# Autodesk Inventor assembly: Grid_Of_Piers
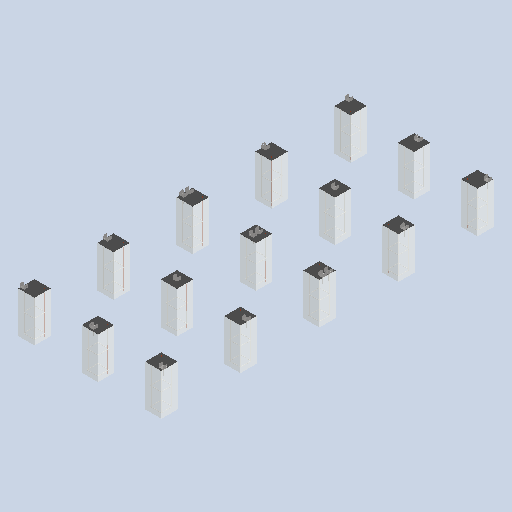
[picture p0: Inventor's stored thumbnail of the model, 512x512]
Saved by Autodesk Inventor 2025.1 (Build 291241020, 241B)
## iProperties
Created: 2024-08-07
Part Number: Grid_Of_Piers
Document SubType Name: Assembly
Designer: Tom
Author: Tom
## Documents named in this file (4)
- C:\Users\Tom\Documents\Inventor\Mobility\Additional_Building\Grid_Of_Piers.iam
- C:\Users\Tom\Documents\Inventor\Mobility\Additional_Building\Pier.iam
- C:\Users\Tom\Documents\Inventor\Mobility\Additional_Building\Saddle_Bracket.ipt
- C:\Users\Tom\Documents\Inventor\Mobility\Additional_Building\Ground_Rod.ipt
## Components (48 placed, 3 different names)
1. Saddle_Bracket:1 — Mate:1, Flush:1, Flush:2
2. Saddle_Bracket:2 — Mate:2, Flush:3, Mate:10
3. Saddle_Bracket:3 — Mate:3, Flush:5, Mate:11
4. Saddle_Bracket:4 — Mate:4, Flush:7, Mate:12
5. Saddle_Bracket:5 — Mate:5, Mate:6, Mate:7
6. Saddle_Bracket:6 — Mate:8, Mate:9, Mate:13
7. Saddle_Bracket:7 — Mate:14, Flush:8, Flush:9
8. Saddle_Bracket:8 — Mate:15, Flush:10, Mate:16
9. Saddle_Bracket:9 — Flush:11, Mate:17, Flush:12
10. Saddle_Bracket:10 — Mate:18, Mate:19, Flush:13
11. Saddle_Bracket:11 — Mate:20, Mate:21, Mate:22
12. Saddle_Bracket:12 — Mate:23, Flush:14, Mate:24
13. Saddle_Bracket:13 — Mate:25, Flush:15, Flush:18
14. Saddle_Bracket:14 — Mate:27, Mate:28, Flush:17
15. Saddle_Bracket:15 — Mate:30, Mate:31, Flush:16
16. Saddle_Bracket:16 — Mate:32, Mate:33, Flush:21
17. Saddle_Bracket:17 — Mate:35, Flush:19, Flush:20
18. Saddle_Bracket:18 — Mate:36, Flush:22, Flush:23
19. Ground_Rod:1 — Flush:24, Tangent:1, Tangent:2
20. Ground_Rod:2 — Flush:25, Tangent:3, Tangent:4
21. Ground_Rod:3 — Flush:26, Tangent:5, Tangent:6
22. Ground_Rod:4 — Flush:27, Mate:40, Mate:41
23. Ground_Rod:5 — Flush:28, Mate:45, Mate:46
24. Ground_Rod:6 — Flush:29, Mate:47, Mate:48
25. Ground_Rod:7 — Flush:30, Mate:53, Mate:54
26. Ground_Rod:8 — Flush:31, Mate:44, Flush:41
27. Ground_Rod:9 — Flush:32, Mate:43, Flush:40
28. Ground_Rod:10 — Flush:33, Tangent:7, Tangent:9, Tangent:10
29. Ground_Rod:11 — Flush:34, Mate:42, Flush:39
30. Ground_Rod:12 — Flush:35, Mate:49, Mate:50
31. Ground_Rod:13 — Flush:36, Mate:51, Mate:52
32. Ground_Rod:14 — Flush:37, Mate:55, Flush:42
33. Ground_Rod:15 — Flush:38, Mate:56, Flush:43
34. Pier:1 [sub-assembly] — Mate:1, Flush:1, Flush:2, Mate:37, Mate:38, Mate:39, Flush:28, Mate:40, Mate:41
35. Pier:2 [sub-assembly] — Mate:2, Flush:3, Mate:10, Flush:27, Tangent:7, Tangent:9, Tangent:10
36. Pier:3 [sub-assembly] — Mate:3, Flush:5, Mate:11, Mate:14, Flush:8, Flush:9, Flush:26, Tangent:5, Tangent:6
37. Pier:4 [sub-assembly] — Mate:15, Flush:10, Mate:16, Flush:25, Tangent:3, Tangent:4
38. Pier:5 [sub-assembly] — Flush:11, Mate:17, Flush:12, Flush:24, Tangent:1, Tangent:2
39. Pier:6 [sub-assembly] — Mate:4, Flush:7, Mate:12, Flush:29, Mate:47, Mate:48
40. Pier:7 [sub-assembly] — Mate:5, Mate:6, Mate:7, Flush:30, Mate:45, Mate:46
41. Pier:8 [sub-assembly] — Mate:8, Mate:9, Mate:13, Mate:18, Mate:19, Flush:13, Flush:31, Mate:44, Flush:41
42. Pier:9 [sub-assembly] — Mate:20, Mate:21, Mate:22, Flush:32, Mate:43, Flush:40
43. Pier:10 [sub-assembly] — Mate:23, Flush:14, Mate:24, Flush:33, Mate:42, Flush:39
44. Pier:11 [sub-assembly] — Mate:25, Flush:15, Flush:18, Flush:38, Mate:56, Flush:43
45. Pier:12 [sub-assembly] — Mate:27, Mate:28, Flush:17, Flush:37, Mate:55, Flush:42
46. Pier:13 [sub-assembly] — Mate:30, Mate:31, Flush:16, Mate:36, Flush:22, Flush:23, Flush:36, Mate:53, Mate:54
47. Pier:14 [sub-assembly] — Mate:32, Mate:33, Flush:21, Flush:35, Mate:51, Mate:52
48. Pier:15 [sub-assembly] — Mate:35, Flush:19, Flush:20, Flush:34, Mate:49, Mate:50
## Component patterns: (15 elements, first: Pier:1)
## Relationships (103: Mate 53, Flush 41, Tangent 9)
- Mate:1: Saddle_Bracket:1 ↔ Pier:1
- Flush:1 (-3.175 mm): Saddle_Bracket:1 ↔ Pier:1
- Flush:2 (38.1 mm): Saddle_Bracket:1 ↔ Pier:1
- Mate:2: Saddle_Bracket:2 ↔ Pier:2
- Flush:3 (-3.175 mm): Saddle_Bracket:2 ↔ Pier:2
- Mate:3: Saddle_Bracket:3 ↔ Pier:3
- Flush:5 (-3.175 mm): Saddle_Bracket:3 ↔ Pier:3
- Mate:4: Saddle_Bracket:4 ↔ Pier:6
- Flush:7 (38.1 mm): Saddle_Bracket:4 ↔ Pier:6
- Mate:5: Saddle_Bracket:5 ↔ Pier:7
- Mate:6: Saddle_Bracket:5 ↔ Pier:7
- Mate:7: Saddle_Bracket:5 ↔ Pier:7
- Mate:8: Saddle_Bracket:6 ↔ Pier:8
- Mate:9: Saddle_Bracket:6 ↔ Pier:8
- Mate:10: Saddle_Bracket:2 ↔ Pier:2
- Mate:11 (19.05 mm): Saddle_Bracket:3 ↔ Pier:3
- Mate:12: Saddle_Bracket:4 ↔ Pier:6
- Mate:13 (19.05 mm): Saddle_Bracket:6 ↔ Pier:8
- Mate:14: Saddle_Bracket:7 ↔ Pier:3
- Flush:8 (-3.175 mm): Saddle_Bracket:7 ↔ Pier:3
- Flush:9 (19.05 mm): Saddle_Bracket:7 ↔ Pier:3
- Mate:15: Saddle_Bracket:8 ↔ Pier:4
- Flush:10 (-3.175 mm): Saddle_Bracket:8 ↔ Pier:4
- Mate:16: Saddle_Bracket:8 ↔ Pier:4
- Flush:11 (38.1 mm): Saddle_Bracket:9 ↔ Pier:5
- Mate:17: Saddle_Bracket:9 ↔ Pier:5
- Flush:12 (-3.175 mm): Saddle_Bracket:9 ↔ Pier:5
- Mate:18: Saddle_Bracket:10 ↔ Pier:8
- Mate:19: Saddle_Bracket:10 ↔ Pier:8
- Flush:13 (19.05 mm): Saddle_Bracket:10 ↔ Pier:8
- Mate:20: Saddle_Bracket:11 ↔ Pier:9
- Mate:21: Saddle_Bracket:11 ↔ Pier:9
- Mate:22: Saddle_Bracket:11 ↔ Pier:9
- Mate:23: Saddle_Bracket:12 ↔ Pier:10
- Flush:14 (38.1 mm): Saddle_Bracket:12 ↔ Pier:10
- Mate:24: Saddle_Bracket:12 ↔ Pier:10
- Mate:25: Saddle_Bracket:13 ↔ Pier:11
- Flush:15 (38.1 mm): Saddle_Bracket:13 ↔ Pier:11
- Mate:27: Saddle_Bracket:14 ↔ Pier:12
- Mate:28: Saddle_Bracket:14 ↔ Pier:12
- Mate:30: Saddle_Bracket:15 ↔ Pier:13
- Mate:31 (19.05 mm): Saddle_Bracket:15 ↔ Pier:13
- Flush:16 (-3.175 mm): Saddle_Bracket:15 ↔ Pier:13
- Flush:17 (-3.175 mm): Saddle_Bracket:14 ↔ Pier:12
- Flush:18 (-3.175 mm): Saddle_Bracket:13 ↔ Pier:11
- Mate:32: Saddle_Bracket:16 ↔ Pier:14
- Mate:33: Saddle_Bracket:16 ↔ Pier:14
- Mate:35: Saddle_Bracket:17 ↔ Pier:15
- Flush:19 (-3.175 mm): Saddle_Bracket:17 ↔ Pier:15
- Flush:20 (38.1 mm): Saddle_Bracket:17 ↔ Pier:15
- Flush:21 (-3.175 mm): Saddle_Bracket:16 ↔ Pier:14
- Mate:36: Saddle_Bracket:18 ↔ Pier:13
- Flush:22 (-3.175 mm): Saddle_Bracket:18 ↔ Pier:13
- Flush:23 (19.05 mm): Saddle_Bracket:18 ↔ Pier:13
- Mate:37: Pier:1
- Mate:38: Pier:1
- Mate:39: Pier:1
- Flush:24 (-12.7 mm): Ground_Rod:1 ↔ Pier:5
- Flush:25 (-12.7 mm): Ground_Rod:2 ↔ Pier:4
- Flush:26 (-12.7 mm): Ground_Rod:3 ↔ Pier:3
- Flush:27 (-12.7 mm): Ground_Rod:4 ↔ Pier:2
- Flush:28 (-12.7 mm): Ground_Rod:5 ↔ Pier:1
- Flush:29 (-12.7 mm): Ground_Rod:6 ↔ Pier:6
- Flush:30 (-12.7 mm): Ground_Rod:7 ↔ Pier:7
- Flush:31 (-12.7 mm): Ground_Rod:8 ↔ Pier:8
- Flush:32 (-12.7 mm): Ground_Rod:9 ↔ Pier:9
- Flush:33 (-12.7 mm): Ground_Rod:10 ↔ Pier:10
- Flush:34 (-12.7 mm): Ground_Rod:11 ↔ Pier:15
- Flush:35 (-12.7 mm): Ground_Rod:12 ↔ Pier:14
- Flush:36 (-12.7 mm): Ground_Rod:13 ↔ Pier:13
- Flush:37 (-12.7 mm): Ground_Rod:14 ↔ Pier:12
- Flush:38 (-12.7 mm): Ground_Rod:15 ↔ Pier:11
- Tangent:1: Ground_Rod:1 ↔ Pier:5
- Tangent:2: Ground_Rod:1 ↔ Pier:5
- Tangent:3: Ground_Rod:2 ↔ Pier:4
- Tangent:4: Ground_Rod:2 ↔ Pier:4
- Tangent:5: Ground_Rod:3 ↔ Pier:3
- Tangent:6: Ground_Rod:3 ↔ Pier:3
- Tangent:7: Ground_Rod:10 ↔ Pier:2
- Tangent:9: Ground_Rod:10 ↔ Pier:2
- Tangent:10: Ground_Rod:10 ↔ Pier:2
- Mate:40 (-69.85 mm): Ground_Rod:4 ↔ Pier:1
- Mate:41 (-69.85 mm): Ground_Rod:4 ↔ Pier:1
- Mate:42 (-69.85 mm): Ground_Rod:11 ↔ Pier:10
- Flush:39 (69.85 mm): Ground_Rod:11 ↔ Pier:10
- Mate:43 (-69.85 mm): Ground_Rod:9 ↔ Pier:9
- Flush:40 (69.85 mm): Ground_Rod:9 ↔ Pier:9
- Mate:44 (-69.85 mm): Ground_Rod:8 ↔ Pier:8
- Flush:41 (69.85 mm): Ground_Rod:8 ↔ Pier:8
- Mate:45 (-69.85 mm): Ground_Rod:5 ↔ Pier:7
- Mate:46 (-69.85 mm): Ground_Rod:5 ↔ Pier:7
- Mate:47 (-69.85 mm): Ground_Rod:6 ↔ Pier:6
- Mate:48 (-69.85 mm): Ground_Rod:6 ↔ Pier:6
- Mate:49 (-69.85 mm): Ground_Rod:12 ↔ Pier:15
- Mate:50 (-69.85 mm): Ground_Rod:12 ↔ Pier:15
- Mate:51 (-69.85 mm): Ground_Rod:13 ↔ Pier:14
- Mate:52 (-69.85 mm): Ground_Rod:13 ↔ Pier:14
- Mate:53 (-69.85 mm): Ground_Rod:7 ↔ Pier:13
- Mate:54 (-69.85 mm): Ground_Rod:7 ↔ Pier:13
- Mate:55 (-69.85 mm): Ground_Rod:14 ↔ Pier:12
- Flush:42 (69.85 mm): Ground_Rod:14 ↔ Pier:12
- Mate:56 (-69.85 mm): Ground_Rod:15 ↔ Pier:11
- Flush:43 (69.85 mm): Ground_Rod:15 ↔ Pier:11
